# Autodesk Inventor assembly: Ensamblaje
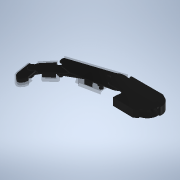
[picture p0: Inventor's stored thumbnail of the model, 180x180]
Saved by Autodesk Inventor 2022 (Build 260153000, 153)
## iProperties
Created: 2022-11-04
Part Number: Ensamblaje
Document SubType Name: Assembly
Designer: Mauricio Guerrero
Author: Mauricio Guerrero
## Documents named in this file (13)
- C:\Users\Griselda Hernandez\Documents\FIME\7mo Semestre\Biomecanica\PIA\PiezasPIA\Ensamblaje.iam
- C:\Users\Griselda Hernandez\Documents\FIME\7mo Semestre\Biomecanica\PIA\PiezasPIA\Pieza4.ipt
- C:\Users\Griselda Hernandez\Documents\FIME\7mo Semestre\Biomecanica\PIA\PiezasPIA\Pieza1.ipt
- C:\Users\Griselda Hernandez\Documents\FIME\7mo Semestre\Biomecanica\PIA\PiezasPIA\Pieza2.ipt
- C:\Users\Griselda Hernandez\Documents\FIME\7mo Semestre\Biomecanica\PIA\PiezasPIA\Pieza3.ipt
- C:\Users\Griselda Hernandez\Documents\FIME\7mo Semestre\Biomecanica\PIA\PiezasPIA\Pieza5.ipt
- C:\Users\Griselda Hernandez\Documents\FIME\7mo Semestre\Biomecanica\PIA\PiezasPIA\Pieza8.ipt
- C:\Users\Griselda Hernandez\Documents\FIME\7mo Semestre\Biomecanica\PIA\PiezasPIA\Pieza9.ipt
- C:\Users\Griselda Hernandez\Documents\FIME\7mo Semestre\Biomecanica\PIA\PiezasPIA\Pieza4_Carcasa.ipt
- C:\Users\Griselda Hernandez\Documents\FIME\7mo Semestre\Biomecanica\PIA\PiezasPIA\Pieza1_Carcasa.ipt
- C:\Users\Griselda Hernandez\Documents\FIME\7mo Semestre\Biomecanica\PIA\PiezasPIA\Pieza2_Carcasa.ipt
- C:\Users\Griselda Hernandez\Documents\FIME\7mo Semestre\Biomecanica\PIA\PiezasPIA\Pieza3_Carcasa.ipt
- C:\Users\Griselda Hernandez\Documents\FIME\7mo Semestre\Biomecanica\PIA\PiezasPIA\Pieza11.ipt
## Components (20 placed, 12 different names)
1. Pieza4:1 — Coincidencia:1, Coincidencia:2, Coincidencia:59, Coincidencia:60, Coincidencia:61, Nivelación:1, Coincidencia:62
2. Pieza1:1 — Coincidencia:1, Coincidencia:2, Coincidencia:3, Coincidencia:4, Coincidencia:14, Coincidencia:15, Coincidencia:24, Coincidencia:39, Coincidencia:48, Coincidencia:49, Coincidencia:50, Coincidencia:51, Coincidencia:52, Coincidencia:55, Coincidencia:56, Coincidencia:63, Nivelación:2, Coincidencia:64
3. Pieza2:1 — Coincidencia:3, Coincidencia:4, Coincidencia:5, Coincidencia:6, Coincidencia:23, Coincidencia:41, Coincidencia:42, Coincidencia:43, Coincidencia:44, Coincidencia:45, Coincidencia:67, Nivelación:4, Coincidencia:68
4. Pieza3:1 — Coincidencia:5, Coincidencia:6, Coincidencia:40, Coincidencia:46, Coincidencia:47, Coincidencia:65, Nivelación:3, Coincidencia:66
5. Pieza5:1 — Coincidencia:14, Coincidencia:15, Coincidencia:22, Coincidencia:53, Coincidencia:54, Coincidencia:57, Coincidencia:58
6. Pieza9:2 — Coincidencia:39, Coincidencia:40, Coincidencia:44
7. Pieza8:2 — Coincidencia:22, Coincidencia:23, Coincidencia:24
8. Pieza11:1 — Coincidencia:59, Coincidencia:60
9. Pieza11:2 — Coincidencia:55, Coincidencia:56
10. Pieza11:3 — Coincidencia:57, Coincidencia:58
11. Pieza11:4 — Coincidencia:49, Coincidencia:50
12. Pieza11:5 — Coincidencia:46, Coincidencia:47
13. Pieza11:6 — Coincidencia:48, Coincidencia:51, Coincidencia:52
14. Pieza11:7 — Coincidencia:43, Coincidencia:45
15. Pieza11:8 — Coincidencia:41, Coincidencia:42
16. Pieza11:9 — Coincidencia:53, Coincidencia:54
17. Pieza4_Carcasa:1 — Coincidencia:61, Nivelación:1, Coincidencia:62
18. Pieza1_Carcasa:1 — Coincidencia:63, Nivelación:2, Coincidencia:64
19. Pieza3_Carcasa:1 — Coincidencia:65, Nivelación:3, Coincidencia:66
20. Pieza2_Carcasa:1 — Coincidencia:67, Nivelación:4, Coincidencia:68
## Relationships (45: Mate 41, Flush 4)
- Coincidencia:1 [Mate]: Pieza4:1 ↔ Pieza1:1
- Coincidencia:2 [Mate]: Pieza4:1 ↔ Pieza1:1
- Coincidencia:3 [Mate]: Pieza1:1 ↔ Pieza2:1
- Coincidencia:4 [Mate]: Pieza1:1 ↔ Pieza2:1
- Coincidencia:5 [Mate]: Pieza2:1 ↔ Pieza3:1
- Coincidencia:6 [Mate]: Pieza2:1 ↔ Pieza3:1
- Coincidencia:14 [Mate]: Pieza1:1 ↔ Pieza5:1
- Coincidencia:15 [Mate]: Pieza1:1 ↔ Pieza5:1
- Coincidencia:22 [Mate]: Pieza5:1 ↔ Pieza8:2
- Coincidencia:23 [Mate]: Pieza2:1 ↔ Pieza8:2
- Coincidencia:24 [Mate]: Pieza1:1 ↔ Pieza8:2
- Coincidencia:39 [Mate]: Pieza1:1 ↔ Pieza9:2
- Coincidencia:40 [Mate]: Pieza3:1 ↔ Pieza9:2
- Coincidencia:41 [Mate]: Pieza2:1 ↔ Pieza11:8
- Coincidencia:42 [Mate]: Pieza2:1 ↔ Pieza11:8
- Coincidencia:43 [Mate]: Pieza2:1 ↔ Pieza11:7
- Coincidencia:44 [Mate]: Pieza2:1 ↔ Pieza9:2
- Coincidencia:45 [Mate]: Pieza2:1 ↔ Pieza11:7
- Coincidencia:46 [Mate]: Pieza3:1 ↔ Pieza11:5
- Coincidencia:47 [Mate]: Pieza3:1 ↔ Pieza11:5
- Coincidencia:48 [Mate]: Pieza1:1 ↔ Pieza11:6
- Coincidencia:49 [Mate]: Pieza1:1 ↔ Pieza11:4
- Coincidencia:50 [Mate]: Pieza1:1 ↔ Pieza11:4
- Coincidencia:51 [Mate]: Pieza1:1 ↔ Pieza11:6
- Coincidencia:52 [Mate]: Pieza1:1 ↔ Pieza11:6
- Coincidencia:53 [Mate]: Pieza5:1 ↔ Pieza11:9
- Coincidencia:54 [Mate]: Pieza5:1 ↔ Pieza11:9
- Coincidencia:55 [Mate]: Pieza1:1 ↔ Pieza11:2
- Coincidencia:56 [Mate]: Pieza1:1 ↔ Pieza11:2
- Coincidencia:57 [Mate]: Pieza5:1 ↔ Pieza11:3
- Coincidencia:58 [Mate]: Pieza5:1 ↔ Pieza11:3
- Coincidencia:59 [Mate]: Pieza4:1 ↔ Pieza11:1
- Coincidencia:60 [Mate]: Pieza4:1 ↔ Pieza11:1
- Coincidencia:61 [Mate]: Pieza4:1 ↔ Pieza4_Carcasa:1
- Nivelación:1 [Flush]: Pieza4:1 ↔ Pieza4_Carcasa:1
- Coincidencia:62 [Mate]: Pieza4:1 ↔ Pieza4_Carcasa:1
- Coincidencia:63 [Mate]: Pieza1:1 ↔ Pieza1_Carcasa:1
- Nivelación:2 [Flush]: Pieza1:1 ↔ Pieza1_Carcasa:1
- Coincidencia:64 [Mate]: Pieza1:1 ↔ Pieza1_Carcasa:1
- Coincidencia:65 [Mate]: Pieza3:1 ↔ Pieza3_Carcasa:1
- Nivelación:3 [Flush]: Pieza3:1 ↔ Pieza3_Carcasa:1
- Coincidencia:66 [Mate]: Pieza3:1 ↔ Pieza3_Carcasa:1
- Coincidencia:67 [Mate]: Pieza2:1 ↔ Pieza2_Carcasa:1
- Nivelación:4 [Flush]: Pieza2:1 ↔ Pieza2_Carcasa:1
- Coincidencia:68 [Mate]: Pieza2:1 ↔ Pieza2_Carcasa:1
